# Autodesk Inventor assembly: fourPmtDetector
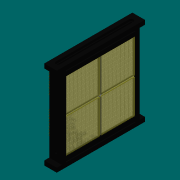
[picture p0: Inventor's stored thumbnail of the model, 180x180]
Saved by Autodesk Inventor 2016 SP1 (Build 200210100, 210)
## iProperties
Created: 2016-04-02
Part Number: fourPmtDetector
Document SubType Name: Assembly
Designer: sawai
Author: sawai
## Documents named in this file (5)
- C:\Users\sawai\OneDrive\projects\modularRICH\detector\fourPmtDetector.iam
- C:\Users\sawai\OneDrive\projects\modularRICH\detector\detectorArray.iam
- C:\Users\sawai\OneDrive\projects\modularRICH\detector\detectorSuppourt.ipt
- C:\Users\sawai\OneDrive\projects\modularRICH\detector\verticalSupourt.ipt
- C:\Users\sawai\OneDrive\projects\modularRICH\detector\horizontalSupourt.ipt
## Components (8 placed, 4 different names)
1. detectorArray:1 [sub-assembly] — Mate:2, Flush:3, Flush:11, Mate:16
2. detectorSuppourt:2 — Mate:2, Flush:3, Mate:3, Flush:5, Flush:6, Mate:4, Symmetry:6
3. verticalSupourt:1 — Mate:3, Flush:5, Flush:7, Flush:8, Flush:9, Mate:11, Symmetry:1, Mate:12, Mate:14, Flush:13
4. verticalSupourt:2 — Flush:6, Mate:4, Flush:7, Mate:10, Symmetry:1
5. horizontalSupourt:1 — Flush:8, Mate:10, Flush:10, Symmetry:3, Symmetry:4, Symmetry:5
6. horizontalSupourt:2 — Flush:9, Mate:11, Flush:10, Symmetry:3, Symmetry:4, Symmetry:5
7. detectorArray:2 [sub-assembly] — Flush:11, Mate:12, Flush:12, Mate:15, Mate:16, Flush:13
8. detectorSuppourt:3 — Flush:12, Mate:14, Mate:15, Symmetry:6
## Relationships (24: Flush 10, Mate 9, Symmetry 5)
- Mate:2: detectorArray:1 ↔ detectorSuppourt:2
- Flush:3: detectorArray:1 ↔ detectorSuppourt:2
- Mate:3: detectorSuppourt:2 ↔ verticalSupourt:1
- Flush:5: detectorSuppourt:2 ↔ verticalSupourt:1
- Flush:6: detectorSuppourt:2 ↔ verticalSupourt:2
- Mate:4: detectorSuppourt:2 ↔ verticalSupourt:2
- Flush:7: verticalSupourt:1 ↔ verticalSupourt:2
- Flush:8: verticalSupourt:1 ↔ horizontalSupourt:1
- Mate:10: verticalSupourt:2 ↔ horizontalSupourt:1
- Flush:9: verticalSupourt:1 ↔ horizontalSupourt:2
- Mate:11: verticalSupourt:1 ↔ horizontalSupourt:2
- Symmetry:1: verticalSupourt:1 ↔ verticalSupourt:2
- Flush:10: horizontalSupourt:1 ↔ horizontalSupourt:2
- Symmetry:3: horizontalSupourt:1 ↔ horizontalSupourt:2
- Symmetry:4: horizontalSupourt:1 ↔ horizontalSupourt:2
- Symmetry:5: horizontalSupourt:1 ↔ horizontalSupourt:2
- Flush:11: detectorArray:1 ↔ detectorArray:2
- Mate:12: verticalSupourt:1 ↔ detectorArray:2
- Flush:12: detectorArray:2 ↔ detectorSuppourt:3
- Mate:14: verticalSupourt:1 ↔ detectorSuppourt:3
- Mate:15: detectorArray:2 ↔ detectorSuppourt:3
- Symmetry:6: detectorSuppourt:2 ↔ detectorSuppourt:3
- Mate:16 (1 mm): detectorArray:1 ↔ detectorArray:2
- Flush:13: verticalSupourt:1 ↔ detectorArray:2
